# Autodesk Inventor assembly: Intake
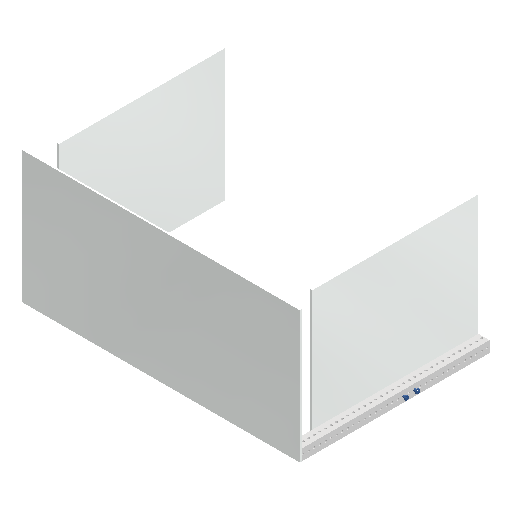
[picture p0: Inventor's stored thumbnail of the model, 512x512]
Saved by Autodesk Inventor 2027.1 (Build 311270010, 270A)
## iProperties
Created: 2026-08-12
Part Number: Intake
Document SubType Name: Assembly
Designer: djair.oliveira
Author: djair.oliveira
## Documents named in this file (6)
- C:\Users\djair.oliveira\Documents\GitHub\MT_2026\CAD\Model C\Intake\Intake.iam
- C:\Users\djair.oliveira\Documents\GitHub\MT_2026\CAD\Model C\Intake\Move - Intake.ipt
- C:\Users\djair.oliveira\Documents\GitHub\MT_2026\CAD\Model C\Intake\Chapa Lateral - Intake.ipt
- C:\Users\djair.oliveira\Documents\GitHub\MT_2026\CAD\Model C\Intake\Suporte Coletor - Intake.ipt
- C:\Users\djair.oliveira\Documents\GitHub\MT_2026\CAD\Model C\Intake\Chapa Frontal - Intake.ipt
- C:\Users\djair.oliveira\Documents\GitHub\MT_2026\CAD\Model C\Intake\Suporte Guia - Intake.ipt
## Components (11 placed, 5 different names)
1. Move - Intake:1 — Alinhado:1, Alinhado:2, Coincidente:2, Alinhado:5, Alinhado:6, Coincidente:6, Coincidente:7, Coincidente:8, Coincidente:9, Coincidente:12, Coincidente:14, Coincidente:21, Coincidente:22
2. Move - Intake:2 — Alinhado:1, Alinhado:2, Coincidente:1, Alinhado:3, Alinhado:4, Coincidente:3, Coincidente:4, Coincidente:5, Coincidente:9, Coincidente:10, Alinhado:7, Alinhado:8, Coincidente:16, Coincidente:17, Coincidente:19, Coincidente:20
3. Chapa Lateral - Intake:1 — Coincidente:2, Alinhado:5, Alinhado:6
4. Chapa Lateral - Intake:2 — Coincidente:1, Alinhado:3, Alinhado:4
5. Suporte Coletor - Intake:1 — Coincidente:3, Coincidente:4, Coincidente:5
6. Suporte Coletor - Intake:2 — Coincidente:6, Coincidente:7, Coincidente:8
7. Chapa Frontal - Intake:1 — Coincidente:10, Alinhado:7, Alinhado:8
8. Suporte Guia - Intake:1 — Coincidente:17, Coincidente:20
9. Suporte Guia - Intake:2 — Coincidente:16, Coincidente:19
10. Suporte Guia - Intake:3 — Coincidente:14, Coincidente:22
11. Suporte Guia - Intake:4 — Coincidente:12, Coincidente:21
## Relationships (26: Mate 18, Flush 8)
- Alinhado:1 [Flush]: Move - Intake:1 ↔ Move - Intake:2
- Alinhado:2 [Flush]: Move - Intake:1 ↔ Move - Intake:2
- Coincidente:1 [Mate]: Move - Intake:2 ↔ Chapa Lateral - Intake:2
- Coincidente:2 [Mate]: Move - Intake:1 ↔ Chapa Lateral - Intake:1
- Alinhado:3 [Flush]: Move - Intake:2 ↔ Chapa Lateral - Intake:2
- Alinhado:4 [Flush]: Move - Intake:2 ↔ Chapa Lateral - Intake:2
- Alinhado:5 [Flush]: Move - Intake:1 ↔ Chapa Lateral - Intake:1
- Alinhado:6 [Flush]: Move - Intake:1 ↔ Chapa Lateral - Intake:1
- Coincidente:3 [Mate]: Move - Intake:2 ↔ Suporte Coletor - Intake:1
- Coincidente:4 [Mate]: Move - Intake:2 ↔ Suporte Coletor - Intake:1
- Coincidente:5 [Mate]: Move - Intake:2 ↔ Suporte Coletor - Intake:1
- Coincidente:6 [Mate]: Move - Intake:1 ↔ Suporte Coletor - Intake:2
- Coincidente:7 [Mate]: Move - Intake:1 ↔ Suporte Coletor - Intake:2
- Coincidente:8 [Mate]: Move - Intake:1 ↔ Suporte Coletor - Intake:2
- Coincidente:9 [Mate] (-631.35 mm): Move - Intake:1 ↔ Move - Intake:2
- Coincidente:10 [Mate]: Move - Intake:2 ↔ Chapa Frontal - Intake:1
- Alinhado:7 [Flush]: Move - Intake:2 ↔ Chapa Frontal - Intake:1
- Alinhado:8 [Flush]: Move - Intake:2 ↔ Chapa Frontal - Intake:1
- Coincidente:12 [Mate]: Move - Intake:1 ↔ Suporte Guia - Intake:4
- Coincidente:14 [Mate]: Move - Intake:1 ↔ Suporte Guia - Intake:3
- Coincidente:16 [Mate]: Move - Intake:2 ↔ Suporte Guia - Intake:2
- Coincidente:17 [Mate]: Move - Intake:2 ↔ Suporte Guia - Intake:1
- Coincidente:19 [Mate]: Move - Intake:2 ↔ Suporte Guia - Intake:2
- Coincidente:20 [Mate]: Move - Intake:2 ↔ Suporte Guia - Intake:1
- Coincidente:21 [Mate]: Move - Intake:1 ↔ Suporte Guia - Intake:4
- Coincidente:22 [Mate]: Move - Intake:1 ↔ Suporte Guia - Intake:3
